# Autodesk Inventor assembly: Kegelrad
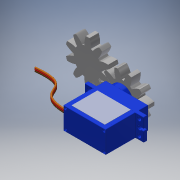
[picture p0: Inventor's stored thumbnail of the model, 180x180]
Saved by Autodesk Inventor 2018 (Build 220112000, 112)
## iProperties
Created: 2018-01-26
Part Number: Kegelrad
Material: Generisch
Document SubType Name: Assembly
Designer: gchri
Author: gchri
## Documents named in this file (3)
- C:\Users\gchri\OneDrive\Development\RTW\03_Konstruktion\StirnradUNDServo.iam
- C:\Users\gchri\Downloads\Servo HXT900 Micro.iam
- C:\Users\gchri\OneDrive\Development\RTW\03_Konstruktion\Kegelrad\Konstruktions-Assistent\Stirnräder2.iam
## Components (2 placed, 2 different names)
1. Servo HXT900 Micro:1 [sub-assembly] — Starr:1
2. Stirnräder:1 [sub-assembly] — Starr:1
## Relationships (1: WeldJoint 1)
- Starr:1 [WeldJoint]: Servo HXT900 Micro:1 ↔ Stirnräder:1
